# Autodesk Inventor assembly: LED-Ring_Camera-Arm
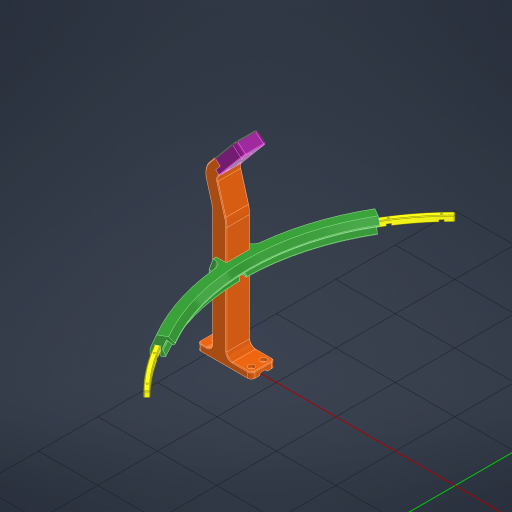
[picture p0: Inventor's stored thumbnail of the model, 512x512]
Saved by Autodesk Inventor 2023.2 (Build 272271030, 271C)
## iProperties
Created: 2023-02-19
Part Number: LED-Ring_Camera-Arm
Document SubType Name: Assembly
Designer: Stefan
Author: Stefan
## Documents named in this file (7)
- C:\Users\Stefan\OneDrive\Inventor\AutoDarts\LED-Ring_Camera-Arm.iam
- C:\Users\Stefan\OneDrive\Inventor\AutoDarts\LED-Ring_Foot_v2.ipt
- C:\Users\Stefan\OneDrive\Inventor\AutoDarts\LED-Ring_Camera-Housing.ipt
- C:\Users\Stefan\OneDrive\Inventor\AutoDarts\LED-Ring_Mount_v2.ipt
- C:\Users\Stefan\OneDrive\Inventor\AutoDarts\LED-Ring_Connector_v2.ipt
- C:\Users\Stefan\OneDrive\Inventor\AutoDarts\Viewcone.ipt
- C:\Users\Stefan\OneDrive\Inventor\AutoDarts\LED-Ring_Camera-Cover.ipt
## Components (7 placed, 6 different names)
1. LED-Ring_Foot_v2:1 — Fluchtend:1, Fluchtend:2, Fluchtend:3, Passend:1, Passend:2, Passend:3, Passend:4, Passend:5, Passend:6
2. LED-Ring_Camera-Housing:1 — Passend:1, Passend:2, Passend:3, Passend:13, Passend:14, Passend:15, Passend:16
3. LED-Ring_Mount_v2:1 — Passend:4, Passend:5, Passend:6, Passend:7, Passend:8, Passend:9, Passend:10, Passend:11, Passend:12
4. LED-Ring_Connector_v2:1 — Passend:7, Passend:8, Passend:9
5. LED-Ring_Connector_v2:2 — Passend:10, Passend:11, Passend:12
6. Viewcone:1 — Passend:13
7. LED-Ring_Camera-Cover:1 — Passend:14, Passend:15, Passend:16
## Relationships (19: Mate 16, Flush 3)
- Fluchtend:1 [Flush]: LED-Ring_Foot_v2:1
- Fluchtend:2 [Flush]: LED-Ring_Foot_v2:1
- Fluchtend:3 [Flush] (-10 mm): LED-Ring_Foot_v2:1
- Passend:1 [Mate]: LED-Ring_Foot_v2:1 ↔ LED-Ring_Camera-Housing:1
- Passend:2 [Mate]: LED-Ring_Foot_v2:1 ↔ LED-Ring_Camera-Housing:1
- Passend:3 [Mate]: LED-Ring_Foot_v2:1 ↔ LED-Ring_Camera-Housing:1
- Passend:4 [Mate]: LED-Ring_Foot_v2:1 ↔ LED-Ring_Mount_v2:1
- Passend:5 [Mate]: LED-Ring_Foot_v2:1 ↔ LED-Ring_Mount_v2:1
- Passend:6 [Mate]: LED-Ring_Foot_v2:1 ↔ LED-Ring_Mount_v2:1
- Passend:7 [Mate]: LED-Ring_Mount_v2:1 ↔ LED-Ring_Connector_v2:1
- Passend:8 [Mate]: LED-Ring_Mount_v2:1 ↔ LED-Ring_Connector_v2:1
- Passend:9 [Mate]: LED-Ring_Mount_v2:1 ↔ LED-Ring_Connector_v2:1
- Passend:10 [Mate]: LED-Ring_Mount_v2:1 ↔ LED-Ring_Connector_v2:2
- Passend:11 [Mate]: LED-Ring_Mount_v2:1 ↔ LED-Ring_Connector_v2:2
- Passend:12 [Mate]: LED-Ring_Mount_v2:1 ↔ LED-Ring_Connector_v2:2
- Passend:13 [Mate]: LED-Ring_Camera-Housing:1 ↔ Viewcone:1
- Passend:14 [Mate]: LED-Ring_Camera-Housing:1 ↔ LED-Ring_Camera-Cover:1
- Passend:15 [Mate]: LED-Ring_Camera-Housing:1 ↔ LED-Ring_Camera-Cover:1
- Passend:16 [Mate]: LED-Ring_Camera-Housing:1 ↔ LED-Ring_Camera-Cover:1
